# Autodesk Inventor assembly: Assembly3
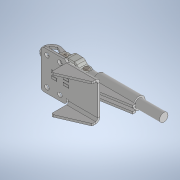
[picture p0: Inventor's stored thumbnail of the model, 180x180]
Saved by Autodesk Inventor 2021.2 (Build 252289000, 289)
## iProperties
Created: 2026-06-23
Part Number: Assembly3
Document SubType Name: Assembly
Designer: nelso
Author: nelso
## Documents named in this file (8)
- C:\Users\nelso\Desktop\Soporte paciente espinografia\Soporte Paciente Espinografia\Workspaces\Workspace\Assembly3.iam
- C:\Users\nelso\Desktop\Soporte paciente espinografia\Soporte Paciente Espinografia\Workspaces\Workspace\base_cuerpo_chapa.ipt
- C:\Users\nelso\Desktop\Soporte paciente espinografia\Soporte Paciente Espinografia\Workspaces\Workspace\cuerpo_chapa.ipt
- C:\Users\nelso\Desktop\Soporte paciente espinografia\Soporte Paciente Espinografia\Workspaces\Workspace\Part4.ipt
- C:\Users\nelso\Desktop\Soporte paciente espinografia\Soporte Paciente Espinografia\Workspaces\Workspace\palanca2.ipt
- C:\Users\nelso\Desktop\Soporte paciente espinografia\Soporte Paciente Espinografia\Workspaces\Workspace\Remache 1.ipt
- C:\Users\nelso\Desktop\Soporte paciente espinografia\Soporte Paciente Espinografia\Workspaces\Workspace\Viela GH-304-305-CM.ipt
- C:\Users\nelso\Desktop\Soporte paciente espinografia\Soporte Paciente Espinografia\Workspaces\Workspace\vastago.ipt
## Components (10 placed, 7 different names)
1. base_cuerpo_chapa:1 — Mate:5, Flush:2, Mate:11, Mate:13, Mate:35, Mate:46, Mate:58
2. cuerpo_chapa:1 — Mate:13, Flush:3, Mate:46, Flush:5
3. cuerpo_chapa:2 — Mate:11, Flush:4, Tangent:1, Mate:58
4. palanca2:1 — Mate:34, Mate:38, Mate:49
5. Remache 1:2 — Mate:22, Mate:48, Mate:49, Mate:50, Mate:55, Mate:56
6. Remache 1:3 — Mate:51, Mate:52, Mate:53, Mate:54
7. Viela GH-304-305-CM:1 — Mate:22, Mate:47, Mate:48, Mate:53, Mate:56
8. Viela GH-304-305-CM:2 — Mate:50, Mate:51, Mate:54, Mate:55
9. vastago:1 — Mate:41, Mate:52, Mate:57, Flush:6
10. Part4:1 — Mate:33, Mate:40, Tangent:1, Flush:5, Mate:57, Flush:6
## Relationships (29: Mate 23, Flush 5, Tangent 1)
- Mate:5: base_cuerpo_chapa:1
- Flush:2: base_cuerpo_chapa:1
- Mate:11: base_cuerpo_chapa:1 ↔ cuerpo_chapa:2
- Mate:13: base_cuerpo_chapa:1 ↔ cuerpo_chapa:1
- Mate:22: Remache 1:2 ↔ Viela GH-304-305-CM:1
- Mate:33: Part4:1
- Mate:34: palanca2:1
- Flush:3 (4 mm): cuerpo_chapa:1
- Mate:35: base_cuerpo_chapa:1
- Flush:4 (-4 mm): cuerpo_chapa:2
- Mate:38: palanca2:1
- Mate:40: Part4:1
- Tangent:1: cuerpo_chapa:2 ↔ Part4:1
- Mate:41: vastago:1
- Mate:46: base_cuerpo_chapa:1 ↔ cuerpo_chapa:1
- Mate:47 (7.5 mm): Viela GH-304-305-CM:1
- Mate:48: Remache 1:2 ↔ Viela GH-304-305-CM:1
- Mate:49: palanca2:1 ↔ Remache 1:2
- Mate:50: Remache 1:2 ↔ Viela GH-304-305-CM:2
- Mate:51: Remache 1:3 ↔ Viela GH-304-305-CM:2
- Mate:52: Remache 1:3 ↔ vastago:1
- Mate:53: Remache 1:3 ↔ Viela GH-304-305-CM:1
- Mate:54: Remache 1:3 ↔ Viela GH-304-305-CM:2
- Mate:55: Remache 1:2 ↔ Viela GH-304-305-CM:2
- Mate:56: Remache 1:2 ↔ Viela GH-304-305-CM:1
- Flush:5: cuerpo_chapa:1 ↔ Part4:1
- Mate:57: vastago:1 ↔ Part4:1
- Flush:6 (-18 mm): vastago:1 ↔ Part4:1
- Mate:58: base_cuerpo_chapa:1 ↔ cuerpo_chapa:2
